# Autodesk Inventor assembly: arm_assembly
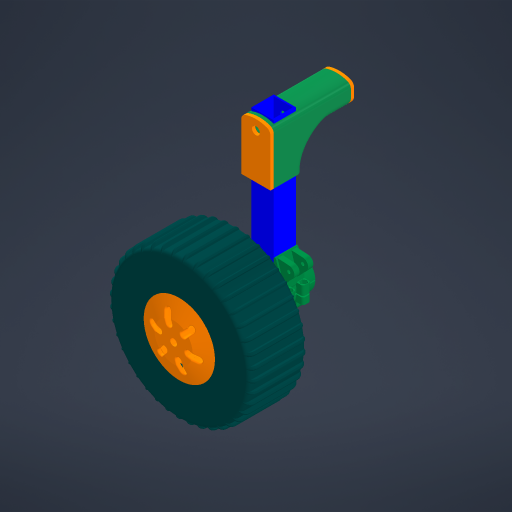
[picture p0: Inventor's stored thumbnail of the model, 512x512]
Saved by Autodesk Inventor 2024 (Build 280153000, 153)
## iProperties
Created: 2023-09-26
Part Number: arm_assembly
Document SubType Name: Assembly
Designer: user
Author: user
## Documents named in this file (6)
- D:\Docs\Robot\3d_v2\machine_body\arm_assembly_l.iam
- D:\Docs\Robot\3d_v2\default_components\motor.ipt
- D:\Docs\Robot\3d_v2\machine_body\arm_assembly\wheel_assembly.iam
- D:\Docs\Robot\3d_v2\machine_body\arm_assembly\arm_holder.iam
- D:\Docs\Robot\3d_v2\base\arm.ipt
- D:\Docs\Robot\3d_v2\machine_body\arm_assembly\motor_holder_l.ipt
## Components (5 placed, 5 different names)
1. motor:1 — Вставка:5, Вставка:6
2. wheel_assembly:1 [sub-assembly] — Вставка:6
3. arm_holder:1 [sub-assembly] — Совмещение:1, Вставка:4
4. arm:1 — Совмещение:1, Вставка:4, Заподлицо:1, Заподлицо:2, Совмещение:2, Совмещение:3, Совмещение:4, Совмещение:5
5. motor_holder_l:1 — Совмещение:3, Совмещение:4, Совмещение:5, Вставка:5
## Relationships (10: Mate 5, Insert 3, Flush 2)
- Совмещение:1 [Mate]: arm_holder:1 ↔ arm:1
- Вставка:4 [Insert]: arm_holder:1 ↔ arm:1
- Заподлицо:1 [Flush]: arm:1
- Заподлицо:2 [Flush]: arm:1
- Совмещение:2 [Mate]: arm:1
- Совмещение:3 [Mate]: arm:1 ↔ motor_holder_l:1
- Совмещение:4 [Mate]: arm:1 ↔ motor_holder_l:1
- Совмещение:5 [Mate]: arm:1 ↔ motor_holder_l:1
- Вставка:5 [Insert] (5 mm): motor:1 ↔ motor_holder_l:1
- Вставка:6 [Insert]: motor:1 ↔ wheel_assembly:1
